# Autodesk Inventor assembly: HoleMountAssembly
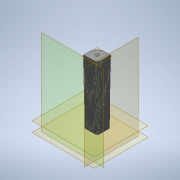
[picture p0: Inventor's stored thumbnail of the model, 180x180]
Saved by Autodesk Inventor 2022 (Build 260153000, 153)
## iProperties
Created: 2021-11-10
Part Number: HoleMountAssembly
Document SubType Name: Assembly
Designer: Viktor
Author: Viktor
## Documents named in this file (3)
- C:\Users\Viktor\Documents\GitHub\MARV-Hardware-Mechanical\InventorProjects\MCU - Marv Communication Unit\HoleMountAssembly.iam
- C:\Users\Viktor\Documents\GitHub\MARV-Hardware-Mechanical\InventorProjects\MCU - Marv Communication Unit\boxAfterMesh.ipt
- C:\Users\Viktor\Documents\GitHub\MARV-Hardware-Mechanical\InventorProjects\MCU - Marv Communication Unit\HoleMount.ipt
## Components (2 placed, 2 different names)
1. boxAfterMesh:1
2. HoleMount:1 — Mate:1, Mate:2, Flush:1
## Relationships (3: Mate 2, Flush 1)
- Mate:1 (17 mm): HoleMount:1
- Mate:2 (8 mm): HoleMount:1
- Flush:1 (11 mm): HoleMount:1
